# Autodesk Inventor assembly: connection_18
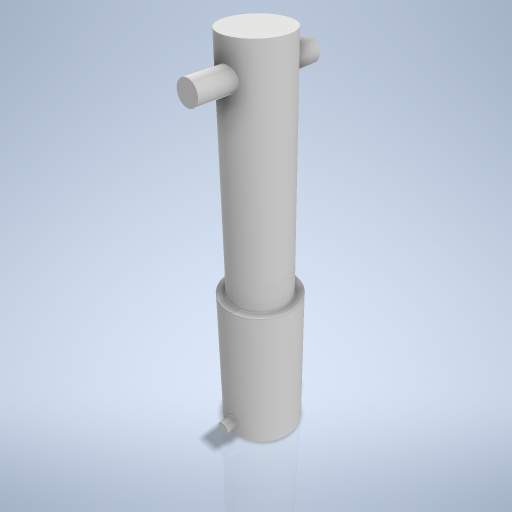
[picture p0: Inventor's stored thumbnail of the model, 512x512]
Saved by Autodesk Inventor 2024.2 (Build 282272000, 272)
## iProperties
Created: 2024-05-05
Part Number: connection_18
Document SubType Name: Assembly
Designer: Fabri
Author: Fabri
## Documents named in this file (4)
- C:\Users\Fabri\Documents\Inventor\stirlingEngine\connection_18.iam
- C:\Users\Fabri\Documents\Inventor\stirlingEngine\18.ipt
- C:\Users\Fabri\Documents\Inventor\stirlingEngine\19,1.ipt
- C:\Users\Fabri\Documents\Inventor\stirlingEngine\18,1.ipt
## Components (3 placed, 3 different names)
1. 18:1 — Passend:1, Drehbar:1, Passend:2, Drehbar:2
2. 19,1:1 — Passend:1, Drehbar:1
3. 18,1:1 — Passend:2, Drehbar:2
## Relationships (4: Mate 2, RevoluteJoint 2)
- Passend:1 [Mate]: 18:1 ↔ 19,1:1
- Drehbar:1 [RevoluteJoint] (-40 mm): 18:1 ↔ 19,1:1
- Passend:2 [Mate]: 18:1 ↔ 18,1:1
- Drehbar:2 [RevoluteJoint] (-42 mm): 18:1 ↔ 18,1:1
